# Autodesk Inventor assembly: final project assembly 3
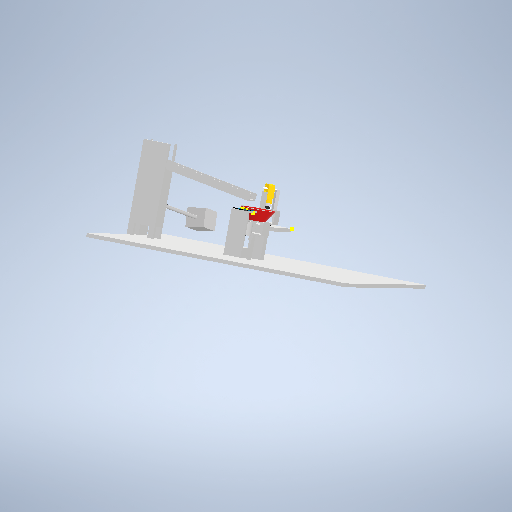
[picture p0: Inventor's stored thumbnail of the model, 512x512]
Saved by Autodesk Inventor 2025.3 (Build 293356000, 356)
## iProperties
Created: 2026-06-07
Part Number: final project assembly 3
Document SubType Name: Assembly
Designer: Hi-Tech
Author: Hi-Tech
## Documents named in this file (18)
- C:\Users\Hi-Tech\New folder (7)\final project assembly 3.iam
- C:\Users\Hi-Tech\New folder (7)\sorting.ipt
- C:\Users\Hi-Tech\New folder (7)\slide shooting.ipt
- C:\Users\Hi-Tech\New folder (7)\lifting arm.ipt
- C:\Users\Hi-Tech\New folder (7)\part 8.ipt
- C:\Users\Hi-Tech\New folder (7)\Part2.ipt
- C:\Users\Hi-Tech\New folder (7)\Part3.ipt
- C:\Users\Hi-Tech\New folder (7)\project slide.ipt
- C:\Users\Hi-Tech\New folder (7)\shooting x.ipt
- C:\Users\Hi-Tech\New folder (7)\cup slide.ipt
- C:\Users\Hi-Tech\New folder (7)\Color_sensor_PCB.ipt
- C:\Users\Hi-Tech\New folder (7)\tcs3200-color-sensor-module-1.snapshot.4\assembly board.ipt
- C:\Users\Hi-Tech\New folder (7)\tcs3200-color-sensor-module-1.snapshot.4\mg90s.ipt
- C:\Users\Hi-Tech\New folder (7)\tcs3200-color-sensor-module-1.snapshot.4\assembly lifting part.ipt
- C:\Users\Hi-Tech\New folder (7)\tcs3200-color-sensor-module-1.snapshot.4\dc motor.iam
- C:\Users\Hi-Tech\New folder (7)\liftng table 2.ipt
- C:\Users\Hi-Tech\New folder (7)\shooting arm.ipt
- C:\Users\Hi-Tech\New folder (7)\shotinjg slide 2.ipt
## Components (20 placed, 17 different names)
1. sorting:1 — Mate:1, Mate:2, Rigid:1, Mate:6, Mate:7, Rigid:10
2. slide shooting:1 — Rigid:2
3. lifting arm:1 — Mate:3
4. part 8:1 — Rigid:2, Rigid:3, Rigid:11
5. Part2:1 — Rotational:1
6. Part3:1
7. Part3:2
8. Part3:3
9. project slide:1 — Mate:4
10. shooting x:1 — Rigid:5, Rigid:9, Mate:5
11. cup slide:1 — Rigid:3
12. Color_sensor_PCB:1 — Mate:1, Mate:2
13. assembly board:1 — Rigid:6, Rigid:7, Rigid:9, Mate:6, Mate:7, Rigid:10, Rigid:11
14. mg90s:1 — Rigid:1, Rotational:1
15. mg90s:2 — Rigid:4, Mate:3
16. assembly lifting part:1 — Rigid:4, Rigid:6
17. dc motor:1 [sub-assembly] — Rigid:5, Rigid:8
18. liftng table 2:1 — Rigid:7, Mate:4
19. shooting arm:1 — Rigid:8
20. shotinjg slide 2:1 — Mate:5
## Relationships (19: WeldJoint 11, Mate 7, RevoluteJoint 1)
- Mate:1: sorting:1 ↔ Color_sensor_PCB:1
- Mate:2: sorting:1 ↔ Color_sensor_PCB:1
- Rigid:1 [WeldJoint]: sorting:1 ↔ mg90s:1
- Rotational:1 [RevoluteJoint]: Part2:1 ↔ mg90s:1
- Rigid:2 [WeldJoint]: slide shooting:1 ↔ part 8:1
- Rigid:3 [WeldJoint] (-35 mm): part 8:1 ↔ cup slide:1
- Rigid:4 [WeldJoint]: mg90s:2 ↔ assembly lifting part:1
- Mate:3: lifting arm:1 ↔ mg90s:2
- Rigid:5 [WeldJoint]: shooting x:1 ↔ dc motor:1
- Rigid:6 [WeldJoint] (-150 mm): assembly board:1 ↔ assembly lifting part:1
- Rigid:7 [WeldJoint]: assembly board:1 ↔ liftng table 2:1
- Mate:4: project slide:1 ↔ liftng table 2:1
- Rigid:8 [WeldJoint]: dc motor:1 ↔ shooting arm:1
- Rigid:9 [WeldJoint]: shooting x:1 ↔ assembly board:1
- Mate:5: shooting x:1 ↔ shotinjg slide 2:1
- Mate:6: sorting:1 ↔ assembly board:1
- Mate:7: sorting:1 ↔ assembly board:1
- Rigid:10 [WeldJoint]: sorting:1 ↔ assembly board:1
- Rigid:11 [WeldJoint]: part 8:1 ↔ assembly board:1
## Named parameters: Finish1_Area = 156.861
note: some values were not read from the file. Shown as the stored number, unit unknown: "Finish1_Area".
